# Autodesk Inventor assembly: !Arm
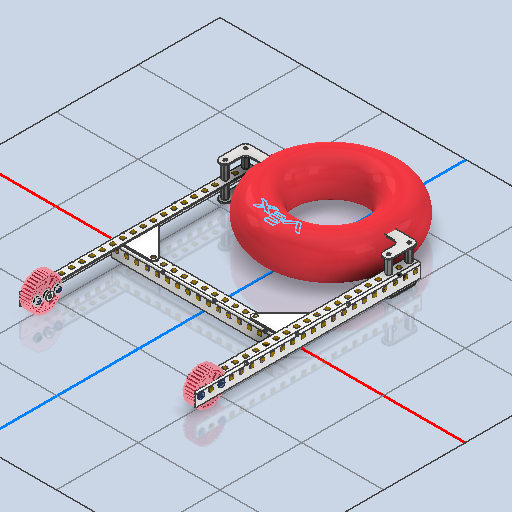
[picture p0: Inventor's stored thumbnail of the model, 512x512]
Saved by Autodesk Inventor 2026 (Build 300175000, 175)
## iProperties
Created: 2025-04-06
Part Number: !Arm
Document SubType Name: Assembly
Designer: avere
Author: avere
## Documents named in this file (24)
- C:\Users\avere\OneDrive\Documents\VEX-CAD\V5-CAD\Lady Brown\Arm\!Arm.iam
- C:\Users\avere\OneDrive\Documents\VEX-CAD\VEX-CAD-Inventor\Structure\C Channel\Aluminum 1x3x1 Half Thick Cut\Alu C Half Thick 1x3x1x22.ipt
- C:\Users\avere\OneDrive\Documents\VEX-CAD\VEX-CAD-Inventor\Motion\Gears\HS Gear\HS 36T Gear, No Insert.iam
- C:\Users\avere\OneDrive\Documents\VEX-CAD\VEX-CAD-Inventor\Motion\Gears\HS Gear.iam
- C:\Users\avere\OneDrive\Documents\VEX-CAD\VEX-CAD-Inventor\Structure\Hardware\Screw Steel - Star\SScrew Star Smooth .750.ipt
- C:\Users\avere\OneDrive\Documents\VEX-CAD\VEX-CAD-Inventor\Structure\Hardware\Screw Steel - Star.ipt
- C:\Users\avere\OneDrive\Documents\VEX-CAD\VEX-CAD-Inventor\Structure\Hardware\Nut Nylon\Nut Nylon - Black.ipt
- C:\Users\avere\OneDrive\Documents\VEX-CAD\VEX-CAD-Inventor\Structure\Hardware\Nut Nylon.ipt
- C:\Users\avere\OneDrive\Documents\VEX-CAD\V5-CAD\Lady Brown\Arm\Alu C Half Thick 1x3x1x22 Mirrored.ipt
- C:\Users\avere\OneDrive\Documents\VEX-CAD\VEX-CAD-Inventor\Structure\C Channel\Aluminum 1x3x1 Half Thick Cut\Alu C Half Thick 1x3x1x17.ipt
- C:\Users\avere\OneDrive\Documents\VEX-CAD\V5-CAD\Lady Brown\Arm\Custom Parts\Triangle Gusset.ipt
- C:\Users\avere\OneDrive\Documents\VEX-CAD\V5-CAD\Lady Brown\Arm\Custom Parts\Magazine Gusset.ipt
- C:\Users\avere\OneDrive\Documents\VEX-CAD\VEX-CAD-Inventor\Structure\Standoff\Standoff .75.ipt
- C:\Users\avere\OneDrive\Documents\VEX-CAD\VEX-CAD-Inventor\Structure\Standoff.ipt
- C:\Users\avere\OneDrive\Documents\VEX-CAD\V5-CAD\Lady Brown\Arm\Custom Parts\Magazine Gusset mirrored.ipt
- C:\Users\avere\OneDrive\Documents\VEX-CAD\VEX-CAD-Inventor\Motion\Spacers\Washer Teflon\TWasher .375 OD x .03125.ipt
- C:\Users\avere\OneDrive\Documents\VEX-CAD\VEX-CAD-Inventor\Motion\Spacers\Washer Teflon.ipt
- C:\Users\avere\OneDrive\Documents\VEX-CAD\VEX-CAD-Inventor\Motion\Spacers\Washer Steel\SWasher .375 OD x .015625.ipt
- C:\Users\avere\OneDrive\Documents\VEX-CAD\VEX-CAD-Inventor\Motion\Spacers\Washer Steel.ipt
- C:\Users\avere\OneDrive\Documents\VEX-CAD\VEX-CAD-Inventor\Motion\Spacers\Spacer Nylon .375 OD\NSpacer .375 OD x .375.ipt
- C:\Users\avere\OneDrive\Documents\VEX-CAD\VEX-CAD-Inventor\Motion\Spacers\Spacer Nylon .375 OD.ipt
- C:\Users\avere\OneDrive\Documents\VEX-CAD\VEX-CAD-Inventor\Motion\Spacers\Spacer Nylon .375 OD\NSpacer .375 OD x .125.ipt
- C:\Users\avere\OneDrive\Documents\VEX-CAD\VEX-CAD-Inventor\Motion\Spacers\Washer Teflon\TWasher .375 OD x .04000.ipt
- C:\Users\avere\OneDrive\Documents\VEX-CAD\VEX-CAD-Inventor\Game Objects\High Stakes\Rings\Red Ring.ipt
## Components (34 placed, 16 different names)
1. Alu C Half Thick 1x3x1x22:1 — Mate:1, Mate:2, Flush:1, Insert:1, Mate:3, Angle:1, Insert:2, Mate:7, Insert:9, Insert:10, Insert:12, Insert:14
2. HS 36T Gear, No Insert:1 [sub-assembly] — Insert:1, Mate:3, Insert:3, Insert:21
3. Alu C Half Thick 1x3x1x22 Mirrored:1 — Angle:2, Flush:2, Mate:4, Mate:5, Mate:6, Insert:4, Insert:5, Insert:7, Insert:8
4. HS 36T Gear, No Insert:2 [sub-assembly] — Mate:6, Insert:4, Insert:6, Insert:24
5. Alu C Half Thick 1x3x1x17:1 — Insert:7, Mate:7, Mate:8
6. Triangle Gusset:1 — Insert:8, Mate:8
7. Triangle Gusset:2
8. Magazine Gusset:1 — Insert:11, Mate:11
9. Standoff .75:1 — Insert:10, Insert:11
10. Standoff .75:2 — Insert:9
11. Magazine Gusset:2 — Insert:13, Insert:15
12. Standoff .75:3 — Insert:14, Insert:15
13. Standoff .75:4 — Insert:12, Insert:13
14. Magazine Gusset mirrored:1 — Insert:16
15. Standoff .75:5 — Insert:16
16. Standoff .75:6
17. Magazine Gusset mirrored:2 — Insert:17, Insert:18
18. Standoff .75:7 — Insert:17
19. Standoff .75:8 — Insert:18
20. TWasher .375 OD x .03125:1 — Insert:19, Insert:20
21. SWasher .375 OD x .015625:1 — Insert:19
22. NSpacer .375 OD x .375:1 — Insert:20, Insert:21
23. TWasher .375 OD x .03125:2 — Insert:22
24. NSpacer .375 OD x .125:2 — Insert:23, Insert:24
25. TWasher .375 OD x .04000:3 — Insert:22, Insert:23
26. Red Ring:1 — Mate:9, Mate:10, Mate:11
27. SScrew Star Smooth .750:1 — Insert:2
28. Nut Nylon - Black:1 — Insert:3
29. SScrew Star Smooth .750:2
30. Nut Nylon - Black:2
31. SScrew Star Smooth .750:3 — Insert:5
32. Nut Nylon - Black:3 — Insert:6
33. SScrew Star Smooth .750:4
34. Nut Nylon - Black:4
## Component patterns: (2 elements, first: SScrew Star Smooth .750:1 + Nut Nylon - Black:1), (2 elements, first: SScrew Star Smooth .750:3 + Nut Nylon - Black:3)
## Relationships (39: Insert 24, Mate 11, Flush 2, Angle 2)
- Mate:1 (101.6 mm): Alu C Half Thick 1x3x1x22:1
- Mate:2: Alu C Half Thick 1x3x1x22:1
- Flush:1 (-139.7 mm): Alu C Half Thick 1x3x1x22:1
- Insert:1: Alu C Half Thick 1x3x1x22:1 ↔ HS 36T Gear, No Insert:1
- Mate:3: Alu C Half Thick 1x3x1x22:1 ↔ HS 36T Gear, No Insert:1
- Angle:1 (0 deg): Alu C Half Thick 1x3x1x22:1
- Insert:2: Alu C Half Thick 1x3x1x22:1 ↔ SScrew Star Smooth .750:1
- Insert:3: HS 36T Gear, No Insert:1 ↔ Nut Nylon - Black:1
- Angle:2 (0 deg): Alu C Half Thick 1x3x1x22 Mirrored:1
- Flush:2 (-139.7 mm): Alu C Half Thick 1x3x1x22 Mirrored:1
- Mate:4: Alu C Half Thick 1x3x1x22 Mirrored:1
- Mate:5 (-101.6 mm): Alu C Half Thick 1x3x1x22 Mirrored:1
- Mate:6: Alu C Half Thick 1x3x1x22 Mirrored:1 ↔ HS 36T Gear, No Insert:2
- Insert:4: Alu C Half Thick 1x3x1x22 Mirrored:1 ↔ HS 36T Gear, No Insert:2
- Insert:5: Alu C Half Thick 1x3x1x22 Mirrored:1 ↔ SScrew Star Smooth .750:3
- Insert:6: HS 36T Gear, No Insert:2 ↔ Nut Nylon - Black:3
- Insert:7 (1.5875 mm): Alu C Half Thick 1x3x1x22 Mirrored:1 ↔ Alu C Half Thick 1x3x1x17:1
- Mate:7: Alu C Half Thick 1x3x1x22:1 ↔ Alu C Half Thick 1x3x1x17:1
- Insert:8: Alu C Half Thick 1x3x1x22 Mirrored:1 ↔ Triangle Gusset:1
- Mate:8: Alu C Half Thick 1x3x1x17:1 ↔ Triangle Gusset:1
- Insert:9: Alu C Half Thick 1x3x1x22:1 ↔ Standoff .75:2
- Insert:10: Alu C Half Thick 1x3x1x22:1 ↔ Standoff .75:1
- Insert:11: Magazine Gusset:1 ↔ Standoff .75:1
- Insert:12: Alu C Half Thick 1x3x1x22:1 ↔ Standoff .75:4
- Insert:13: Magazine Gusset:2 ↔ Standoff .75:4
- Insert:14: Alu C Half Thick 1x3x1x22:1 ↔ Standoff .75:3
- Insert:15: Magazine Gusset:2 ↔ Standoff .75:3
- Insert:16: Magazine Gusset mirrored:1 ↔ Standoff .75:5
- Insert:17: Magazine Gusset mirrored:2 ↔ Standoff .75:7
- Insert:18: Magazine Gusset mirrored:2 ↔ Standoff .75:8
- Insert:19: TWasher .375 OD x .03125:1 ↔ SWasher .375 OD x .015625:1
- Insert:20: TWasher .375 OD x .03125:1 ↔ NSpacer .375 OD x .375:1
- Insert:21: HS 36T Gear, No Insert:1 ↔ NSpacer .375 OD x .375:1
- Insert:22: TWasher .375 OD x .03125:2 ↔ TWasher .375 OD x .04000:3
- Insert:23: NSpacer .375 OD x .125:2 ↔ TWasher .375 OD x .04000:3
- Insert:24: HS 36T Gear, No Insert:2 ↔ NSpacer .375 OD x .125:2
- Mate:9: Red Ring:1
- Mate:10 (6.35 mm): Red Ring:1
- Mate:11: Magazine Gusset:1 ↔ Red Ring:1
